# Autodesk Inventor assembly: フィールド
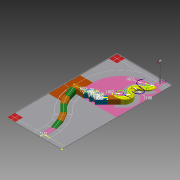
[picture p0: Inventor's stored thumbnail of the model, 180x180]
Saved by Autodesk Inventor 2015 (Build 190159000, 159)
## iProperties
Created: 2015-08-24
Part Number: フィールド
Document SubType Name: Assembly
Designer: nobuhiro
Author: nobuhiro
## Documents named in this file (19)
- C:\Users\陽生\Downloads\島_フィールド\フィールド.iam
- C:\Users\陽生\Downloads\島_フィールド\フィールド.ipt
- C:\Users\陽生\Downloads\島_フィールド\Slope 1.ipt
- C:\Users\陽生\Downloads\島_フィールド\Slope 2.ipt
- C:\Users\陽生\Downloads\島_フィールド\Hill 1.ipt
- C:\Users\陽生\Downloads\島_フィールド\Hill 2.ipt
- C:\Users\陽生\Downloads\島_フィールド\Slope 3.ipt
- C:\Users\陽生\Downloads\島_フィールド\River 1_赤.ipt
- C:\Users\陽生\Downloads\島_フィールド\Hill 3_赤.ipt
- C:\Users\陽生\Downloads\島_フィールド\River 2_赤.ipt
- C:\Users\陽生\Downloads\島_フィールド\River 3_赤.ipt
- C:\Users\陽生\Downloads\島_フィールド\Highland_赤.ipt
- C:\Users\陽生\Downloads\島_フィールド\Island.ipt
- C:\Users\陽生\Downloads\島_フィールド\Pole Base.ipt
- C:\Users\陽生\Downloads\島_フィールド\Wind Turbine Pole.ipt
- C:\Users\陽生\Downloads\島_フィールド\Wind Trubin Engine.ipt
- C:\Users\陽生\Downloads\島_フィールド\Wind Turbine Propeller.ipt
- C:\Users\陽生\Downloads\島_フィールド\Down Hill_赤2.ipt
- C:\Users\陽生\Downloads\島_フィールド\Wind Trubin Turbine Base.ipt
## Components (21 placed, 18 different names)
1. フィールド:1 — メイト:1, メイト:4, メイト:5, メイト:10, メイト:13, メイト:21, メイト:45, メイト:28, メイト:31, メイト:33, メイト:36, メイト:39, メイト:46, メイト:55, メイト:57, メイト:58, メイト:61
2. Slope 1:1 — メイト:1, メイト:6, メイト:7, メイト:21, メイト:45
3. Slope 2:1 — メイト:4, メイト:8, メイト:9, メイト:25, メイト:26
4. Hill 1:1 — メイト:5, メイト:6, メイト:7, メイト:8, メイト:9
5. Hill 2:1 — メイト:10, メイト:23, メイト:24, メイト:25, メイト:26
6. Slope 3:1 — メイト:13, メイト:23, メイト:24, メイト:27, メイト:29
7. River 1_赤:1 — メイト:30, メイト:31, メイト:32, メイト:34, メイト:35, メイト:50, メイト:54
8. Hill 3_赤:1 — メイト:27, メイト:28, メイト:29, メイト:30, メイト:32
9. River 2_赤:1 — メイト:33, メイト:34, メイト:35, メイト:37, メイト:38, メイト:48, メイト:49, メイト:51, メイト:53
10. River 3_赤:1 — メイト:36, メイト:37, メイト:38, メイト:40, メイト:41, メイト:47, メイト:52
11. Highland_赤:1 — メイト:39, メイト:40, メイト:41, メイト:62, フラッシュ:64
12. Island:1 — フラッシュ:1, メイト:49, メイト:50
13. Island:2 — フラッシュ:1, フラッシュ:2, メイト:52, メイト:53
14. Island:3 — フラッシュ:2, フラッシュ:3, メイト:46, メイト:47, メイト:48
15. Island:4 — フラッシュ:3, メイト:51, メイト:54
16. Pole Base:1 — メイト:55, 挿入:1, メイト:57, メイト:58, メイト:59
17. Wind Turbine Pole:1 — 挿入:1, フラッシュ:4, メイト:59, 挿入:3, メイト:63
18. Wind Trubin Engine:1 — メイト:56, フラッシュ:65, フラッシュ:66, 挿入:2, フラッシュ:4
19. Wind Turbine Propeller:1 — 挿入:2
20. Down Hill_赤2:1 — メイト:61, メイト:62, フラッシュ:64
21. Wind Trubin Turbine Base:1 — 挿入:3, メイト:63, メイト:56, フラッシュ:65, フラッシュ:66
## Relationships (57: Mate 47, Flush 7, Insert 3)
- メイト:1 [Mate]: フィールド:1 ↔ Slope 1:1
- メイト:4 [Mate]: フィールド:1 ↔ Slope 2:1
- メイト:5 [Mate]: フィールド:1 ↔ Hill 1:1
- メイト:6 [Mate]: Slope 1:1 ↔ Hill 1:1
- メイト:7 [Mate]: Slope 1:1 ↔ Hill 1:1
- メイト:8 [Mate]: Slope 2:1 ↔ Hill 1:1
- メイト:9 [Mate]: Slope 2:1 ↔ Hill 1:1
- メイト:10 [Mate]: フィールド:1 ↔ Hill 2:1
- メイト:13 [Mate]: フィールド:1 ↔ Slope 3:1
- メイト:21 [Mate]: フィールド:1 ↔ Slope 1:1
- メイト:45 [Mate]: フィールド:1 ↔ Slope 1:1
- メイト:23 [Mate]: Hill 2:1 ↔ Slope 3:1
- メイト:24 [Mate]: Hill 2:1 ↔ Slope 3:1
- メイト:25 [Mate]: Slope 2:1 ↔ Hill 2:1
- メイト:26 [Mate]: Slope 2:1 ↔ Hill 2:1
- メイト:27 [Mate]: Slope 3:1 ↔ Hill 3_赤:1
- メイト:28 [Mate]: フィールド:1 ↔ Hill 3_赤:1
- メイト:29 [Mate]: Slope 3:1 ↔ Hill 3_赤:1
- メイト:30 [Mate]: River 1_赤:1 ↔ Hill 3_赤:1
- メイト:31 [Mate]: フィールド:1 ↔ River 1_赤:1
- メイト:32 [Mate]: River 1_赤:1 ↔ Hill 3_赤:1
- メイト:33 [Mate]: フィールド:1 ↔ River 2_赤:1
- メイト:34 [Mate]: River 1_赤:1 ↔ River 2_赤:1
- メイト:35 [Mate]: River 1_赤:1 ↔ River 2_赤:1
- メイト:36 [Mate]: フィールド:1 ↔ River 3_赤:1
- メイト:37 [Mate]: River 2_赤:1 ↔ River 3_赤:1
- メイト:38 [Mate]: River 2_赤:1 ↔ River 3_赤:1
- メイト:39 [Mate]: フィールド:1 ↔ Highland_赤:1
- メイト:40 [Mate]: River 3_赤:1 ↔ Highland_赤:1
- メイト:41 [Mate]: River 3_赤:1 ↔ Highland_赤:1
- フラッシュ:1 [Flush]: Island:1 ↔ Island:2
- フラッシュ:2 [Flush]: Island:2 ↔ Island:3
- フラッシュ:3 [Flush]: Island:3 ↔ Island:4
- メイト:46 [Mate]: フィールド:1 ↔ Island:3
- メイト:47 [Mate]: River 3_赤:1 ↔ Island:3
- メイト:48 [Mate]: River 2_赤:1 ↔ Island:3
- メイト:49 [Mate]: River 2_赤:1 ↔ Island:1
- メイト:50 [Mate]: River 1_赤:1 ↔ Island:1
- メイト:51 [Mate]: River 2_赤:1 ↔ Island:4
- メイト:52 [Mate]: River 3_赤:1 ↔ Island:2
- メイト:53 [Mate]: River 2_赤:1 ↔ Island:2
- メイト:54 [Mate]: River 1_赤:1 ↔ Island:4
- メイト:55 [Mate]: フィールド:1 ↔ Pole Base:1
- 挿入:1 [Insert]: Pole Base:1 ↔ Wind Turbine Pole:1
- メイト:56 [Mate]: Wind Trubin Engine:1 ↔ Wind Trubin Turbine Base:1
- フラッシュ:65 [Flush]: Wind Trubin Engine:1 ↔ Wind Trubin Turbine Base:1
- フラッシュ:66 [Flush] (-50 mm): Wind Trubin Engine:1 ↔ Wind Trubin Turbine Base:1
- 挿入:2 [Insert]: Wind Trubin Engine:1 ↔ Wind Turbine Propeller:1
- メイト:57 [Mate]: フィールド:1 ↔ Pole Base:1
- メイト:58 [Mate]: フィールド:1 ↔ Pole Base:1
- フラッシュ:4 [Flush]: Wind Turbine Pole:1 ↔ Wind Trubin Engine:1
- メイト:59 [Mate]: Pole Base:1 ↔ Wind Turbine Pole:1
- メイト:61 [Mate]: フィールド:1 ↔ Down Hill_赤2:1
- メイト:62 [Mate]: Highland_赤:1 ↔ Down Hill_赤2:1
- フラッシュ:64 [Flush]: Highland_赤:1 ↔ Down Hill_赤2:1
- 挿入:3 [Insert]: Wind Turbine Pole:1 ↔ Wind Trubin Turbine Base:1
- メイト:63 [Mate]: Wind Turbine Pole:1 ↔ Wind Trubin Turbine Base:1
